# Autodesk Inventor assembly: Угловой v5
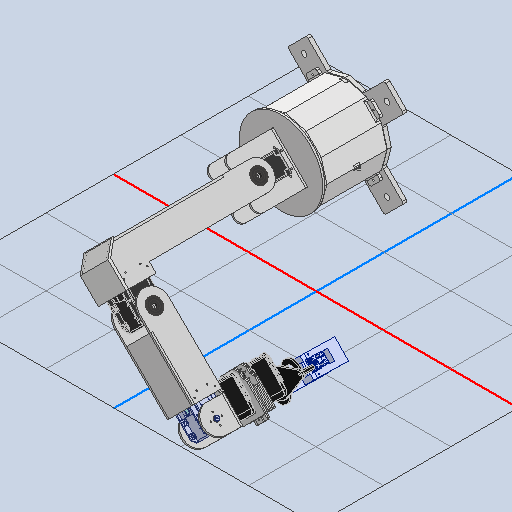
[picture p0: Inventor's stored thumbnail of the model, 512x512]
Saved by Autodesk Inventor 2022 (Build 260153000, 153)
## iProperties
Created: 2022-11-16
Part Number: Угловой v5
Document SubType Name: Assembly
Designer: Petrov Ivan
Author: Petrov Ivan
## Documents named in this file (23)
- D:\IVAN\Ivan_desktop\Kvantorium\Projects\YouBotRobot\design\Манипулятор AR\Угловой v5.iam
- D:\IVAN\Ivan_desktop\Kvantorium\Projects\YouBotRobot\design\Манипулятор AR\Днище.ipt
- D:\IVAN\Ivan_desktop\Kvantorium\Projects\YouBotRobot\design\Манипулятор AR\28Tyy.ipt
- D:\IVAN\Ivan_desktop\Kvantorium\Projects\YouBotRobot\design\Манипулятор AR\Шайба 2.ipt
- D:\IVAN\Ivan_desktop\Kvantorium\Projects\YouBotRobot\design\Манипулятор AR\Вал.ipt
- D:\IVAN\Ivan_desktop\Kvantorium\Projects\YouBotRobot\design\Манипулятор AR\Шайба1.ipt
- D:\IVAN\Ivan_desktop\Kvantorium\Projects\YouBotRobot\design\Манипулятор AR\Деталь8.ipt
- D:\IVAN\Ivan_desktop\Kvantorium\Projects\YouBotRobot\design\Манипулятор AR\snr_ucf201_0.ipt
- D:\IVAN\Ivan_desktop\Kvantorium\Projects\YouBotRobot\design\Манипулятор AR\Кожух.ipt
- D:\IVAN\Ivan_desktop\Kvantorium\Projects\YouBotRobot\design\Манипулятор AR\Стол.ipt
- D:\IVAN\Ivan_desktop\Kvantorium\Projects\YouBotRobot\design\Манипулятор AR\Сборка над столом.iam
- D:\IVAN\Ivan_desktop\Kvantorium\Projects\YouBotRobot\design\Манипулятор AR\MX-64T.ipt
- D:\IVAN\Ivan_desktop\Kvantorium\Projects\YouBotRobot\design\Манипулятор AR\Сборка длинное плечо.iam
- D:\IVAN\Ivan_desktop\Kvantorium\Projects\YouBotRobot\design\Манипулятор AR\Переходник на 64 new.ipt
- D:\IVAN\Ivan_desktop\Kvantorium\Projects\YouBotRobot\design\Манипулятор AR\Сборка среднее плечо.iam
- D:\IVAN\Ivan_desktop\Kvantorium\Projects\YouBotRobot\design\Манипулятор AR\Переходник на 28.ipt
- D:\IVAN\Ivan_desktop\Kvantorium\Projects\YouBotRobot\design\Манипулятор AR\Сборка 28 на18.iam
- D:\IVAN\Ivan_desktop\Kvantorium\Projects\YouBotRobot\design\Манипулятор AR\AX-18A.ipt
- D:\IVAN\Ivan_desktop\Kvantorium\Projects\YouBotRobot\design\Манипулятор AR\Съем1.ipt
- D:\IVAN\Ivan_desktop\Kvantorium\Projects\YouBotRobot\design\Манипулятор AR\Сборка съем.iam
- D:\IVAN\Ivan_desktop\Kvantorium\Projects\YouBotRobot\design\Манипулятор AR\Сборка клешни.iam
- D:\IVAN\Ivan_desktop\Kvantorium\Projects\YouBotRobot\design\Манипулятор AR\3d printed Gripper v4 (1).ipt
- D:\IVAN\Ivan_desktop\Kvantorium\Projects\YouBotRobot\design\Манипулятор AR\Подшипник.ipt
## Components (29 placed, 22 different names)
1. Днище.ipt:1 — Совмещение:1, Совмещение:2, Совмещение:3, Совмещение:7, Совмещение:8, Совмещение:9, Заподлицо:1, Заподлицо:2, Совмещение:19, Угол:3
2. 28Tyy.ipt:1 — Совмещение:7, Совмещение:8, Совмещение:9, Совмещение:10, Совмещение:11
3. Шайба 2.ipt:1 — Совмещение:10, Совмещение:11, Совмещение:12, Совмещение:13
4. Вал.ipt:1 — Совмещение:12, Совмещение:13, Совмещение:14, Совмещение:15
5. Шайба1.ipt:1 — Совмещение:14, Совмещение:15, Совмещение:16, Совмещение:17, Совмещение:18
6. Деталь8.ipt:1 — Совмещение:1, Совмещение:2, Совмещение:3, Совмещение:4, Совмещение:5, Совмещение:6
7. snr_ucf201_0.ipt:1 — Совмещение:4, Совмещение:5, Совмещение:6
8. Кожух.ipt:1 — Заподлицо:1, Заподлицо:2, Совмещение:19
9. Стол.ipt:1 — Совмещение:16, Совмещение:17, Совмещение:18, Совмещение:20, Совмещение:21, Совмещение:22
10. Сборка над столом.iam:1 [sub-assembly] — Совмещение:20, Совмещение:21, Совмещение:22, Совмещение:23, Совмещение:24, Совмещение:25, Угол:2, Угол:3
11. MX-64T.ipt:1 — Совмещение:23, Совмещение:24, Совмещение:25, Совмещение:27, Совмещение:29
12. Сборка длинное плечо.iam:1 [sub-assembly] — Заподлицо:3, Совмещение:26, Совмещение:27, Совмещение:28, Совмещение:29, Совмещение:30, Совмещение:31, Совмещение:32, Угол:2
13. Переходник на 64 new.ipt:1 — Совмещение:30, Совмещение:31, Совмещение:32, Совмещение:33, Угол:1, Угол:4
14. Сборка среднее плечо.iam:1 [sub-assembly] — Заподлицо:4, Совмещение:34, Совмещение:35, Совмещение:36, Угол:4, Совмещение:37, Совмещение:38, Совмещение:39, Совмещение:41, Совмещение:42
15. Переходник на 28.ipt:1 — Совмещение:37, Совмещение:38, Совмещение:39, Совмещение:40
16. Сборка 28 на18.iam:1 [sub-assembly] — Заподлицо:5, Совмещение:43, Совмещение:44, Совмещение:45, Совмещение:46, Совмещение:47, Совмещение:48
17. AX-18A.ipt:1 — Совмещение:46, Совмещение:47, Совмещение:48, Совмещение:52, Совмещение:53, Совмещение:54, Совмещение:55, Совмещение:56, Совмещение:57
18. Съем1.ipt:1 — Совмещение:49, Совмещение:50, Совмещение:51, Совмещение:52, Совмещение:53
19. Сборка съем.iam:1 [sub-assembly] — Совмещение:56, Совмещение:57, Совмещение:58, Совмещение:59, Совмещение:60
20. Сборка клешни.iam:1 [sub-assembly] — Совмещение:63, Совмещение:64, Угол:6
21. 3d printed Gripper v4 (1).ipt:1 — Совмещение:61, Совмещение:62, Угол:5
22. Подшипник.ipt:1 — Заподлицо:5, Совмещение:43
23. MX-64T.ipt:2 — Совмещение:28, Совмещение:33, Угол:1, Совмещение:35, Совмещение:36
24. 28Tyy.ipt:2 — Совмещение:40, Совмещение:41, Совмещение:42, Совмещение:44, Совмещение:45
25. Съем1.ipt:2 — Совмещение:49, Совмещение:50, Совмещение:51, Совмещение:54, Совмещение:55
26. AX-18A.ipt:2 — Совмещение:58, Совмещение:59, Совмещение:60, Совмещение:61, Совмещение:62, Угол:5, Совмещение:63, Совмещение:64, Угол:6
27. Кожух.ipt:2
28. Подшипник.ipt:2 — Заподлицо:4, Совмещение:34
29. Подшипник.ipt:3 — Заподлицо:3, Совмещение:26
## Relationships (75: Mate 64, Angle 6, Flush 5)
- Совмещение:1 [Mate]: Днище.ipt:1 ↔ Деталь8.ipt:1
- Совмещение:2 [Mate]: Днище.ipt:1 ↔ Деталь8.ipt:1
- Совмещение:3 [Mate]: Днище.ipt:1 ↔ Деталь8.ipt:1
- Совмещение:4 [Mate]: Деталь8.ipt:1 ↔ snr_ucf201_0.ipt:1
- Совмещение:5 [Mate]: Деталь8.ipt:1 ↔ snr_ucf201_0.ipt:1
- Совмещение:6 [Mate]: Деталь8.ipt:1 ↔ snr_ucf201_0.ipt:1
- Совмещение:7 [Mate]: Днище.ipt:1 ↔ 28Tyy.ipt:1
- Совмещение:8 [Mate]: Днище.ipt:1 ↔ 28Tyy.ipt:1
- Совмещение:9 [Mate]: Днище.ipt:1 ↔ 28Tyy.ipt:1
- Совмещение:10 [Mate] (3 mm): 28Tyy.ipt:1 ↔ Шайба 2.ipt:1
- Совмещение:11 [Mate]: 28Tyy.ipt:1 ↔ Шайба 2.ipt:1
- Совмещение:12 [Mate]: Шайба 2.ipt:1 ↔ Вал.ipt:1
- Совмещение:13 [Mate]: Шайба 2.ipt:1 ↔ Вал.ipt:1
- Совмещение:14 [Mate]: Вал.ipt:1 ↔ Шайба1.ipt:1
- Совмещение:15 [Mate]: Вал.ipt:1 ↔ Шайба1.ipt:1
- Совмещение:16 [Mate]: Шайба1.ipt:1 ↔ Стол.ipt:1
- Совмещение:17 [Mate]: Шайба1.ipt:1 ↔ Стол.ipt:1
- Совмещение:18 [Mate]: Шайба1.ipt:1 ↔ Стол.ipt:1
- Заподлицо:1 [Flush]: Днище.ipt:1 ↔ Кожух.ipt:1
- Заподлицо:2 [Flush]: Днище.ipt:1 ↔ Кожух.ipt:1
- Совмещение:19 [Mate]: Днище.ipt:1 ↔ Кожух.ipt:1
- Совмещение:20 [Mate]: Стол.ipt:1 ↔ Сборка над столом.iam:1
- Совмещение:21 [Mate]: Стол.ipt:1 ↔ Сборка над столом.iam:1
- Совмещение:22 [Mate]: Стол.ipt:1 ↔ Сборка над столом.iam:1
- Совмещение:23 [Mate]: Сборка над столом.iam:1 ↔ MX-64T.ipt:1
- Совмещение:24 [Mate]: Сборка над столом.iam:1 ↔ MX-64T.ipt:1
- Совмещение:25 [Mate]: Сборка над столом.iam:1 ↔ MX-64T.ipt:1
- Заподлицо:3 [Flush] (-1 mm): Сборка длинное плечо.iam:1 ↔ Подшипник.ipt:3
- Совмещение:26 [Mate]: Сборка длинное плечо.iam:1 ↔ Подшипник.ipt:3
- Совмещение:27 [Mate]: MX-64T.ipt:1 ↔ Сборка длинное плечо.iam:1
- Совмещение:28 [Mate]: Сборка длинное плечо.iam:1 ↔ MX-64T.ipt:2
- Совмещение:29 [Mate]: MX-64T.ipt:1 ↔ Сборка длинное плечо.iam:1
- Совмещение:30 [Mate]: Сборка длинное плечо.iam:1 ↔ Переходник на 64 new.ipt:1
- Совмещение:31 [Mate]: Сборка длинное плечо.iam:1 ↔ Переходник на 64 new.ipt:1
- Совмещение:32 [Mate]: Сборка длинное плечо.iam:1 ↔ Переходник на 64 new.ipt:1
- Совмещение:33 [Mate]: Переходник на 64 new.ipt:1 ↔ MX-64T.ipt:2
- Угол:1 [Angle] (0 deg): Переходник на 64 new.ipt:1 ↔ MX-64T.ipt:2
- Угол:2 [Angle] (0 deg): Сборка над столом.iam:1 ↔ Сборка длинное плечо.iam:1
- Угол:3 [Angle] (0 deg): Днище.ipt:1 ↔ Сборка над столом.iam:1
- Заподлицо:4 [Flush] (-1 mm): Сборка среднее плечо.iam:1 ↔ Подшипник.ipt:2
- Совмещение:34 [Mate]: Сборка среднее плечо.iam:1 ↔ Подшипник.ipt:2
- Совмещение:35 [Mate]: Сборка среднее плечо.iam:1 ↔ MX-64T.ipt:2
- Совмещение:36 [Mate]: Сборка среднее плечо.iam:1 ↔ MX-64T.ipt:2
- Угол:4 [Angle] (0 deg): Переходник на 64 new.ipt:1 ↔ Сборка среднее плечо.iam:1
- Совмещение:37 [Mate]: Сборка среднее плечо.iam:1 ↔ Переходник на 28.ipt:1
- Совмещение:38 [Mate]: Сборка среднее плечо.iam:1 ↔ Переходник на 28.ipt:1
- Совмещение:39 [Mate]: Сборка среднее плечо.iam:1 ↔ Переходник на 28.ipt:1
- Совмещение:40 [Mate]: Переходник на 28.ipt:1 ↔ 28Tyy.ipt:2
- Совмещение:41 [Mate]: Сборка среднее плечо.iam:1 ↔ 28Tyy.ipt:2
- Совмещение:42 [Mate]: Сборка среднее плечо.iam:1 ↔ 28Tyy.ipt:2
- Заподлицо:5 [Flush]: Сборка 28 на18.iam:1 ↔ Подшипник.ipt:1
- Совмещение:43 [Mate]: Сборка 28 на18.iam:1 ↔ Подшипник.ipt:1
- Совмещение:44 [Mate]: Сборка 28 на18.iam:1 ↔ 28Tyy.ipt:2
- Совмещение:45 [Mate]: Сборка 28 на18.iam:1 ↔ 28Tyy.ipt:2
- Совмещение:46 [Mate]: Сборка 28 на18.iam:1 ↔ AX-18A.ipt:1
- Совмещение:47 [Mate]: Сборка 28 на18.iam:1 ↔ AX-18A.ipt:1
- Совмещение:48 [Mate]: Сборка 28 на18.iam:1 ↔ AX-18A.ipt:1
- Совмещение:49 [Mate]: Съем1.ipt:1 ↔ Съем1.ipt:2
- Совмещение:50 [Mate]: Съем1.ipt:1 ↔ Съем1.ipt:2
- Совмещение:51 [Mate]: Съем1.ipt:1 ↔ Съем1.ipt:2
- Совмещение:52 [Mate]: AX-18A.ipt:1 ↔ Съем1.ipt:1
- Совмещение:53 [Mate]: AX-18A.ipt:1 ↔ Съем1.ipt:1
- Совмещение:54 [Mate]: AX-18A.ipt:1 ↔ Съем1.ipt:2
- Совмещение:55 [Mate]: AX-18A.ipt:1 ↔ Съем1.ipt:2
- Совмещение:56 [Mate]: AX-18A.ipt:1 ↔ Сборка съем.iam:1
- Совмещение:57 [Mate]: AX-18A.ipt:1 ↔ Сборка съем.iam:1
- Совмещение:58 [Mate]: Сборка съем.iam:1 ↔ AX-18A.ipt:2
- Совмещение:59 [Mate]: Сборка съем.iam:1 ↔ AX-18A.ipt:2
- Совмещение:60 [Mate]: Сборка съем.iam:1 ↔ AX-18A.ipt:2
- Совмещение:61 [Mate]: 3d printed Gripper v4 (1).ipt:1 ↔ AX-18A.ipt:2
- Совмещение:62 [Mate]: 3d printed Gripper v4 (1).ipt:1 ↔ AX-18A.ipt:2
- Угол:5 [Angle] (179.9087 deg): 3d printed Gripper v4 (1).ipt:1 ↔ AX-18A.ipt:2
- Совмещение:63 [Mate]: Сборка клешни.iam:1 ↔ AX-18A.ipt:2
- Совмещение:64 [Mate]: Сборка клешни.iam:1 ↔ AX-18A.ipt:2
- Угол:6 [Angle] (0 deg): Сборка клешни.iam:1 ↔ AX-18A.ipt:2
